# Autodesk Inventor assembly: vacuum-resivoir
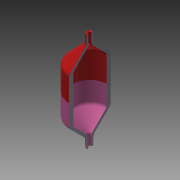
[picture p0: Inventor's stored thumbnail of the model, 180x180]
Saved by Autodesk Inventor 2015 SP2 (Build 190223200, 223)
## iProperties
Created: 2015-12-05
Part Number: vacuum-resivoir
Document SubType Name: Assembly
Designer: caleb
Author: caleb
## Documents named in this file (3)
- C:\cygwin64\home\caleb\3d\vacuum-resivoir\vacuum-resivoir.iam
- C:\cygwin64\home\caleb\3d\vacuum-resivoir\Solid4.ipt
- C:\cygwin64\home\caleb\3d\vacuum-resivoir\Solid5.ipt
## Components (2 placed, 2 different names)
1. Solid4:1 — Mate:1, Mate:2
2. Solid5:1 — Mate:1, Mate:2
## Relationships (2: Mate 2)
- Mate:1: Solid4:1 ↔ Solid5:1
- Mate:2: Solid4:1 ↔ Solid5:1
